# Autodesk Inventor assembly: Assembly7
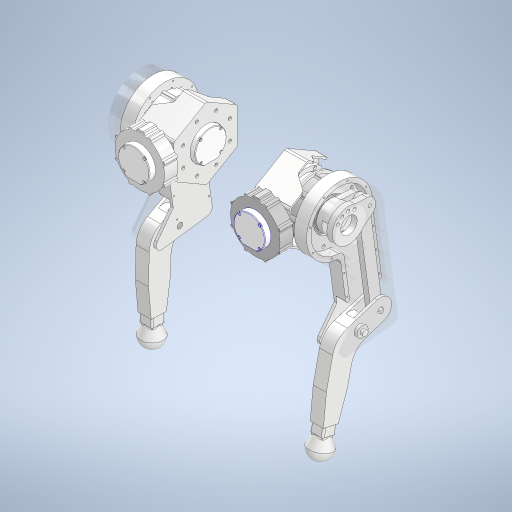
[picture p0: Inventor's stored thumbnail of the model, 512x512]
Saved by Autodesk Inventor 2024.3 (Build 283343000, 343)
## iProperties
Created: 2025-01-16
Part Number: Assembly7
Document SubType Name: Assembly
Designer: 佐藤智貴
Mass: 3127.52 g
Surface Area: 8370.14 cm^2
Volume: 2225.59 cm^3
Density: 1.40525 g/cm^3
Author: 佐藤智貴
## Documents named in this file (42)
- C:\Users\佐藤智貴\OneDrive - Chiba Institute of Technology\ドキュメント\Inventor\Biped_robot\Assembly7.iam
- C:\Users\佐藤智貴\OneDrive - Chiba Institute of Technology\ドキュメント\Inventor\Biped_robot\legparts_06(six).ipt
- C:\Users\佐藤智貴\OneDrive - Chiba Institute of Technology\ドキュメント\Inventor\Biped_robot\legparts_08(six).ipt
- C:\Users\佐藤智貴\OneDrive - Chiba Institute of Technology\ドキュメント\Inventor\Biped_robot\sole05.ipt
- C:\Users\佐藤智貴\OneDrive - Chiba Institute of Technology\ドキュメント\Inventor\Biped_robot\8108-8.iam
- C:\Users\佐藤智貴\OneDrive - Chiba Institute of Technology\ドキュメント\Inventor\Biped_robot\legparts_03(six).ipt
- C:\Users\佐藤智貴\OneDrive - Chiba Institute of Technology\ドキュメント\Inventor\Biped_robot\10mm_bearing.ipt
- C:\Users\佐藤智貴\OneDrive - Chiba Institute of Technology\ドキュメント\Inventor\Biped_robot\legparts_01.ipt
- C:\Users\佐藤智貴\OneDrive - Chiba Institute of Technology\ドキュメント\Inventor\Biped_robot\legparts_10.ipt
- C:\Users\佐藤智貴\OneDrive - Chiba Institute of Technology\ドキュメント\Inventor\Biped_robot\legparts_08(six)_MIR.ipt
- C:\Users\佐藤智貴\OneDrive - Chiba Institute of Technology\ドキュメント\Inventor\Biped_robot\3.5mm_spacer.ipt
- C:\Users\佐藤智貴\OneDrive - Chiba Institute of Technology\ドキュメント\Inventor\Biped_robot\shaft10_30mm.ipt
- C:\Users\佐藤智貴\OneDrive - Chiba Institute of Technology\ドキュメント\Inventor\Biped_robot\shaft10_45mm.ipt
- C:\Users\佐藤智貴\OneDrive - Chiba Institute of Technology\ドキュメント\Inventor\Biped_robot\legparts_02(six).ipt
- C:\Users\佐藤智貴\OneDrive - Chiba Institute of Technology\ドキュメント\Inventor\Biped_robot\legparts_04(six).ipt
- C:\Users\佐藤智貴\OneDrive - Chiba Institute of Technology\ドキュメント\Inventor\Biped_robot\legparts_06(six)_MIR1.ipt
- C:\Users\佐藤智貴\OneDrive - Chiba Institute of Technology\ドキュメント\Inventor\Biped_robot\legparts_08(six)_MIR2.ipt
- C:\Users\佐藤智貴\OneDrive - Chiba Institute of Technology\ドキュメント\Inventor\Biped_robot\sole05_MIR1.ipt
- C:\Users\佐藤智貴\OneDrive - Chiba Institute of Technology\ドキュメント\Inventor\Biped_robot\8108-8_MIR4.iam
- C:\Users\佐藤智貴\OneDrive - Chiba Institute of Technology\ドキュメント\Inventor\Biped_robot\legparts_03(six)_MIR1.ipt
- C:\Users\佐藤智貴\OneDrive - Chiba Institute of Technology\ドキュメント\Inventor\Biped_robot\10mm_bearing_MIR2.ipt
- C:\Users\佐藤智貴\OneDrive - Chiba Institute of Technology\ドキュメント\Inventor\Biped_robot\legparts_01_MIR3.ipt
- C:\Users\佐藤智貴\OneDrive - Chiba Institute of Technology\ドキュメント\Inventor\Biped_robot\legparts_10_MIR1.ipt
- C:\Users\佐藤智貴\OneDrive - Chiba Institute of Technology\ドキュメント\Inventor\Biped_robot\legparts_08(six)_MIR_MIR1.ipt
- C:\Users\佐藤智貴\OneDrive - Chiba Institute of Technology\ドキュメント\Inventor\Biped_robot\3.5mm_spacer_MIR1.ipt
- C:\Users\佐藤智貴\OneDrive - Chiba Institute of Technology\ドキュメント\Inventor\Biped_robot\shaft10_30mm_MIR2.ipt
- C:\Users\佐藤智貴\OneDrive - Chiba Institute of Technology\ドキュメント\Inventor\Biped_robot\shaft10_45mm_MIR1.ipt
- C:\Users\佐藤智貴\OneDrive - Chiba Institute of Technology\ドキュメント\Inventor\Biped_robot\legparts_02(six)_MIR.ipt
- C:\Users\佐藤智貴\OneDrive - Chiba Institute of Technology\ドキュメント\Inventor\Biped_robot\legparts_04(six)_MIR.ipt
- C:\Users\佐藤智貴\OneDrive - Chiba Institute of Technology\ドキュメント\Inventor\Biped_robot\legparts_07(six).ipt
- C:\Users\佐藤智貴\OneDrive - Chiba Institute of Technology\ドキュメント\Inventor\Biped_robot\Assembly7\AIP\FEA\eyqtwukxs.fins
- C:\Users\佐藤智貴\OneDrive - Chiba Institute of Technology\ドキュメント\Inventor\Biped_robot\Assembly7\AIP\FEA\eyqtwukxs.fsat
- C:\Users\佐藤智貴\OneDrive - Chiba Institute of Technology\ドキュメント\Inventor\Biped_robot\Assembly7\AIP\FEA\eyqtwukxs.ftes
- C:\Users\佐藤智貴\OneDrive - Chiba Institute of Technology\ドキュメント\Inventor\Biped_robot\Assembly7\AIP\FEA\eyqtwukxs.fwiz
- C:\Users\佐藤智貴\OneDrive - Chiba Institute of Technology\ドキュメント\Inventor\Biped_robot\Assembly7\AIP\FEA\eyqtwukxt.fins
- C:\Users\佐藤智貴\OneDrive - Chiba Institute of Technology\ドキュメント\Inventor\Biped_robot\Assembly7\AIP\FEA\eyqtwukxt.fsat
- C:\Users\佐藤智貴\OneDrive - Chiba Institute of Technology\ドキュメント\Inventor\Biped_robot\Assembly7\AIP\FEA\eyqtwukxt.ftes
- C:\Users\佐藤智貴\OneDrive - Chiba Institute of Technology\ドキュメント\Inventor\Biped_robot\Assembly7\AIP\FEA\eyqtwukxt.fwiz
- C:\Users\佐藤智貴\OneDrive - Chiba Institute of Technology\ドキュメント\Inventor\Biped_robot\Assembly7\AIP\FEA\eyqtwul5s.fmsh
- C:\Users\佐藤智貴\OneDrive - Chiba Institute of Technology\ドキュメント\Inventor\Biped_robot\Assembly7\AIP\FEA\eyqtwul5t.fres
- C:\Users\佐藤智貴\OneDrive - Chiba Institute of Technology\ドキュメント\Inventor\Biped_robot\Assembly7\AIP\FEA\eyqtwuleo.fmsh
- C:\Users\佐藤智貴\OneDrive - Chiba Institute of Technology\ドキュメント\Inventor\Biped_robot\Assembly7\AIP\FEA\eyqtwulep.fres
## Components (46 placed, 29 different names)
1. legparts_06(six):1 — 挿入:1, メイト:1, 挿入:11, 挿入:12, 挿入:25, 挿入:31, 挿入:32, 挿入:34
2. legparts_08(six):2 — 挿入:2, 挿入:25, 挿入:69, 挿入:70
3. sole05:1 — 挿入:1, メイト:1
4. 8108-8:1 [sub-assembly] — 挿入:2, 挿入:13, 挿入:14, 挿入:75, 挿入:78
5. 8108-8:2 [sub-assembly] — 挿入:112
6. 8108-8:3 [sub-assembly] — 挿入:15, 挿入:27, 挿入:28, 挿入:29, 挿入:30, 挿入:113, 挿入:114
7. legparts_03(six):1 — 挿入:6, 挿入:7, 挿入:9, 挿入:10
8. 10mm_bearing:1 — 挿入:6
9. 10mm_bearing:2 — 挿入:7, 挿入:77
10. 10mm_bearing:3 — 挿入:10, 挿入:11
11. 10mm_bearing:4 — 挿入:9, 挿入:12
12. legparts_01:1 — 挿入:13, 挿入:14, 挿入:15
13. legparts_10:1 — 挿入:29, 挿入:30
14. legparts_10:2 — 挿入:27, 挿入:28
15. legparts_08(six)_MIR:1 — 挿入:35, 挿入:69, 挿入:70
16. 3.5mm_spacer:1 — 挿入:31
17. 3.5mm_spacer:2 — 挿入:32
18. shaft10_30mm:1 — 挿入:76
19. shaft10_30mm:2 — 挿入:34
20. shaft10_45mm:1 — 挿入:35
21. legparts_02(six):1 — 挿入:73, 挿入:74, 挿入:75, 挿入:78
22. legparts_04(six):1 — 挿入:73, 挿入:74, 挿入:76, 挿入:77
23. legparts_06(six)_MIR1:1 — 挿入:79, メイト:2, 挿入:80, 挿入:84, 挿入:86, 挿入:100, 挿入:101, 挿入:102
24. legparts_08(six)_MIR2:1 — 挿入:79, 挿入:81, 挿入:98, 挿入:99
25. sole05_MIR1:1 — メイト:2, 挿入:80
26. 8108-8_MIR4:1 [sub-assembly] — 挿入:81, 挿入:89, 挿入:90, 挿入:104, 挿入:105
27. 8108-8_MIR4:2 [sub-assembly] — 挿入:115, 挿入:116
28. 8108-8_MIR4:3 [sub-assembly] — 挿入:88, 挿入:91, 挿入:92, 挿入:93, 挿入:94, 挿入:117, 挿入:118
29. legparts_03(six)_MIR1:1 — 挿入:82, 挿入:83, 挿入:85, 挿入:87
30. 10mm_bearing_MIR2:1 — 挿入:82
31. 10mm_bearing_MIR2:2 — 挿入:83, 挿入:106
32. 10mm_bearing_MIR2:3 — 挿入:84, 挿入:85
33. 10mm_bearing_MIR2:4 — 挿入:86, 挿入:87
34. legparts_01_MIR3:1 — 挿入:88, 挿入:89, 挿入:90
35. legparts_10_MIR1:1 — 挿入:91, 挿入:92
36. legparts_10_MIR1:2 — 挿入:93, 挿入:94
37. legparts_08(six)_MIR_MIR1:1 — 挿入:98, 挿入:99, 挿入:103
38. 3.5mm_spacer_MIR1:1 — 挿入:100
39. 3.5mm_spacer_MIR1:2 — 挿入:101
40. shaft10_30mm_MIR2:1 — 挿入:107
41. shaft10_30mm_MIR2:2 — 挿入:102
42. shaft10_45mm_MIR1:1 — 挿入:103
43. legparts_02(six)_MIR:1 — 挿入:104, 挿入:105, 挿入:108, 挿入:109
44. legparts_04(six)_MIR:1 — 挿入:106, 挿入:107, 挿入:108, 挿入:109
45. legparts_07(six):1 — 挿入:112, 挿入:113, 挿入:114
46. legparts_07(six):2 — 挿入:115, 挿入:116, 挿入:117, 挿入:118
## Relationships (65: Insert 63, Mate 2)
- 挿入:1 [Insert]: legparts_06(six):1 ↔ sole05:1
- メイト:1 [Mate]: legparts_06(six):1 ↔ sole05:1
- 挿入:2 [Insert]: legparts_08(six):2 ↔ 8108-8:1
- 挿入:6 [Insert]: legparts_03(six):1 ↔ 10mm_bearing:1
- 挿入:7 [Insert]: legparts_03(six):1 ↔ 10mm_bearing:2
- 挿入:9 [Insert]: legparts_03(six):1 ↔ 10mm_bearing:4
- 挿入:10 [Insert]: legparts_03(six):1 ↔ 10mm_bearing:3
- 挿入:11 [Insert]: legparts_06(six):1 ↔ 10mm_bearing:3
- 挿入:12 [Insert]: legparts_06(six):1 ↔ 10mm_bearing:4
- 挿入:13 [Insert]: 8108-8:1 ↔ legparts_01:1
- 挿入:14 [Insert]: 8108-8:1 ↔ legparts_01:1
- 挿入:15 [Insert]: 8108-8:3 ↔ legparts_01:1
- 挿入:25 [Insert] (5.5 mm): legparts_06(six):1 ↔ legparts_08(six):2
- 挿入:27 [Insert]: 8108-8:3 ↔ legparts_10:2
- 挿入:28 [Insert]: 8108-8:3 ↔ legparts_10:2
- 挿入:29 [Insert]: 8108-8:3 ↔ legparts_10:1
- 挿入:30 [Insert]: 8108-8:3 ↔ legparts_10:1
- 挿入:31 [Insert]: legparts_06(six):1 ↔ 3.5mm_spacer:1
- 挿入:32 [Insert]: legparts_06(six):1 ↔ 3.5mm_spacer:2
- 挿入:34 [Insert] (-3 mm): legparts_06(six):1 ↔ shaft10_30mm:2
- 挿入:35 [Insert]: legparts_08(six)_MIR:1 ↔ shaft10_45mm:1
- 挿入:69 [Insert]: legparts_08(six):2 ↔ legparts_08(six)_MIR:1
- 挿入:70 [Insert]: legparts_08(six):2 ↔ legparts_08(six)_MIR:1
- 挿入:73 [Insert]: legparts_02(six):1 ↔ legparts_04(six):1
- 挿入:74 [Insert]: legparts_02(six):1 ↔ legparts_04(six):1
- 挿入:75 [Insert]: 8108-8:1 ↔ legparts_02(six):1
- 挿入:76 [Insert]: shaft10_30mm:1 ↔ legparts_04(six):1
- 挿入:77 [Insert]: 10mm_bearing:2 ↔ legparts_04(six):1
- 挿入:78 [Insert]: 8108-8:1 ↔ legparts_02(six):1
- 挿入:79 [Insert] (5.5 mm): legparts_06(six)_MIR1:1 ↔ legparts_08(six)_MIR2:1
- メイト:2 [Mate]: legparts_06(six)_MIR1:1 ↔ sole05_MIR1:1
- 挿入:80 [Insert]: legparts_06(six)_MIR1:1 ↔ sole05_MIR1:1
- 挿入:81 [Insert]: legparts_08(six)_MIR2:1 ↔ 8108-8_MIR4:1
- 挿入:82 [Insert]: legparts_03(six)_MIR1:1 ↔ 10mm_bearing_MIR2:1
- 挿入:83 [Insert]: legparts_03(six)_MIR1:1 ↔ 10mm_bearing_MIR2:2
- 挿入:84 [Insert]: legparts_06(six)_MIR1:1 ↔ 10mm_bearing_MIR2:3
- 挿入:85 [Insert]: legparts_03(six)_MIR1:1 ↔ 10mm_bearing_MIR2:3
- 挿入:86 [Insert]: legparts_06(six)_MIR1:1 ↔ 10mm_bearing_MIR2:4
- 挿入:87 [Insert]: legparts_03(six)_MIR1:1 ↔ 10mm_bearing_MIR2:4
- 挿入:88 [Insert]: 8108-8_MIR4:3 ↔ legparts_01_MIR3:1
- 挿入:89 [Insert]: 8108-8_MIR4:1 ↔ legparts_01_MIR3:1
- 挿入:90 [Insert]: 8108-8_MIR4:1 ↔ legparts_01_MIR3:1
- 挿入:91 [Insert]: 8108-8_MIR4:3 ↔ legparts_10_MIR1:1
- 挿入:92 [Insert]: 8108-8_MIR4:3 ↔ legparts_10_MIR1:1
- 挿入:93 [Insert]: 8108-8_MIR4:3 ↔ legparts_10_MIR1:2
- 挿入:94 [Insert]: 8108-8_MIR4:3 ↔ legparts_10_MIR1:2
- 挿入:98 [Insert]: legparts_08(six)_MIR2:1 ↔ legparts_08(six)_MIR_MIR1:1
- 挿入:99 [Insert]: legparts_08(six)_MIR2:1 ↔ legparts_08(six)_MIR_MIR1:1
- 挿入:100 [Insert]: legparts_06(six)_MIR1:1 ↔ 3.5mm_spacer_MIR1:1
- 挿入:101 [Insert]: legparts_06(six)_MIR1:1 ↔ 3.5mm_spacer_MIR1:2
- 挿入:102 [Insert] (-3 mm): legparts_06(six)_MIR1:1 ↔ shaft10_30mm_MIR2:2
- 挿入:103 [Insert]: legparts_08(six)_MIR_MIR1:1 ↔ shaft10_45mm_MIR1:1
- 挿入:104 [Insert]: 8108-8_MIR4:1 ↔ legparts_02(six)_MIR:1
- 挿入:105 [Insert]: 8108-8_MIR4:1 ↔ legparts_02(six)_MIR:1
- 挿入:106 [Insert]: 10mm_bearing_MIR2:2 ↔ legparts_04(six)_MIR:1
- 挿入:107 [Insert]: shaft10_30mm_MIR2:1 ↔ legparts_04(six)_MIR:1
- 挿入:108 [Insert]: legparts_02(six)_MIR:1 ↔ legparts_04(six)_MIR:1
- 挿入:109 [Insert]: legparts_02(six)_MIR:1 ↔ legparts_04(six)_MIR:1
- 挿入:112 [Insert]: 8108-8:2 ↔ legparts_07(six):1
- 挿入:113 [Insert]: 8108-8:3 ↔ legparts_07(six):1
- 挿入:114 [Insert]: 8108-8:3 ↔ legparts_07(six):1
- 挿入:115 [Insert]: 8108-8_MIR4:2 ↔ legparts_07(six):2
- 挿入:116 [Insert]: 8108-8_MIR4:2 ↔ legparts_07(six):2
- 挿入:117 [Insert]: 8108-8_MIR4:3 ↔ legparts_07(six):2
- 挿入:118 [Insert]: 8108-8_MIR4:3 ↔ legparts_07(six):2
## Named parameters: sa_0 = 5000, sa_1 = 5000, sa_2 = 0, sa_3 = -6000, sa_4 = 0
note: some values were not read from the file. Shown as the stored number, unit unknown: "sa_0", "sa_1", "sa_2", "sa_3", "sa_4".
